# Autodesk Inventor assembly: сборка серва
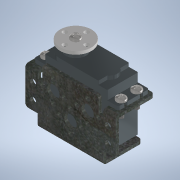
[picture p0: Inventor's stored thumbnail of the model, 180x180]
Saved by Autodesk Inventor 2020.1 (Build 241239000, 239)
## iProperties
Created: 2021-08-12
Part Number: сборка серва
Document SubType Name: Assembly
Designer: User
Author: User
## Documents named in this file (6)
- D:\GitHub\avatar-kvantoriada\3D\сборка серва.iam
- D:\GitHub\avatar-kvantoriada\3D\Деталь4.ipt
- D:\GitHub\avatar-kvantoriada\3D\MG996R.ipt
- D:\GitHub\avatar-kvantoriada\3D\Деталь5.ipt
- C:\Users\User\Documents\Inventor\Content Center Files\R2020\ru-RU\AS 1427(08)\AS 1427 - M3 x 10(6) I.ipt
- C:\Users\User\Documents\Inventor\Content Center Files\R2020\ru-RU\AS 1474(1)\AS 1474 - M3(1).ipt
## Components (12 placed, 5 different names)
1. Деталь4:1 — Жесткий:1, Жесткий:7, Жесткий:8, Жесткий:9, Жесткий:10
2. MG996R:1 — С поворотом:1, Жесткий:1, Жесткий:3, Жесткий:4, Жесткий:5, Жесткий:6
3. Деталь5:1 — С поворотом:1, Жесткий:2
4. AS 1427 Z - метрическая M3 x 10:1 — Жесткий:2
5. AS 1427 Z - метрическая M3 x 10:2 — Жесткий:3
6. AS 1427 Z - метрическая M3 x 10:3 — Жесткий:5
7. AS 1427 Z - метрическая M3 x 10:4 — Жесткий:6
8. AS 1427 Z - метрическая M3 x 10:5 — Жесткий:4
9. AS 1474 - метрическая M3:1 — Жесткий:7
10. AS 1474 - метрическая M3:2 — Жесткий:8
11. AS 1474 - метрическая M3:3 — Жесткий:9
12. AS 1474 - метрическая M3:4 — Жесткий:10
## Relationships (11: WeldJoint 10, RevoluteJoint 1)
- С поворотом:1 [RevoluteJoint]: MG996R:1 ↔ Деталь5:1
- Жесткий:1 [WeldJoint]: Деталь4:1 ↔ MG996R:1
- Жесткий:2 [WeldJoint]: Деталь5:1 ↔ AS 1427 Z - метрическая M3 x 10:1
- Жесткий:3 [WeldJoint]: MG996R:1 ↔ AS 1427 Z - метрическая M3 x 10:2
- Жесткий:4 [WeldJoint]: MG996R:1 ↔ AS 1427 Z - метрическая M3 x 10:5
- Жесткий:5 [WeldJoint]: MG996R:1 ↔ AS 1427 Z - метрическая M3 x 10:3
- Жесткий:6 [WeldJoint]: MG996R:1 ↔ AS 1427 Z - метрическая M3 x 10:4
- Жесткий:7 [WeldJoint]: Деталь4:1 ↔ AS 1474 - метрическая M3:1
- Жесткий:8 [WeldJoint]: Деталь4:1 ↔ AS 1474 - метрическая M3:2
- Жесткий:9 [WeldJoint]: Деталь4:1 ↔ AS 1474 - метрическая M3:3
- Жесткий:10 [WeldJoint]: Деталь4:1 ↔ AS 1474 - метрическая M3:4
